# Autodesk Inventor assembly: AX12
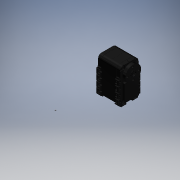
[picture p0: Inventor's stored thumbnail of the model, 180x180]
Saved by Autodesk Inventor 2019 (Build 230136000, 136)
## iProperties
Created: 2010-02-01
Part Number: AX12
Document SubType Name: Assembly
Designer: Andrew
Mass: 42.653 g
Surface Area: 128.735 cm^2
Volume: 42.653 cm^3
Density: 1 g/cm^3
Author: Andrew
## Documents named in this file (4)
- C:\Users\franc\Desktop\EsialRobotik\Mecanique\composants\AX12\AX12.iam
- C:\Users\franc\Desktop\EsialRobotik\Mecanique\composants\AX12\ax12_wheel.ipt
- C:\Users\franc\Desktop\EsialRobotik\Mecanique\composants\AX12\ax12_box.ipt
- C:\Users\franc\Desktop\EsialRobotik\Mecanique\composants\AX12\ax12_cog.ipt
## Components (3 placed, 3 different names)
1. ax12_wheel:1 — Insert:1
2. ax12_box:1 — Insert:1
3. ax12_cog:1
## Relationships (1: Insert 1)
- Insert:1: ax12_wheel:1 ↔ ax12_box:1
